# Autodesk Inventor assembly: Segway
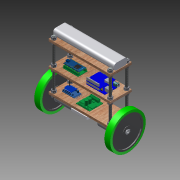
[picture p0: Inventor's stored thumbnail of the model, 180x180]
Saved by Autodesk Inventor 2012 (Build 160160000, 160)
## iProperties
Created: 2012-02-28
Part Number: Segway
Document SubType Name: Assembly
Designer: Grailas
Author: Grailas
## Documents named in this file (24)
- C:\Users\Lauszus\Documents\My Dropbox\Segway\Segway_3DModel\Segway.iam
- C:\Users\Lauszus\Documents\My Dropbox\Segway\Segway_3DModel\plate.ipt
- C:\Users\Lauszus\Documents\My Dropbox\Segway\Segway_3DModel\Screw bar.ipt
- C:\Users\Lauszus\Documents\My Dropbox\Segway\Segway_3DModel\washer.ipt
- C:\Users\Lauszus\Documents\My Dropbox\Segway\Segway_3DModel\bolt.ipt
- C:\Users\Lauszus\Documents\My Dropbox\Segway\Segway_3DModel\Imported Components\uno-assy\uno-assy.iam
- C:\Users\Lauszus\Documents\My Dropbox\Segway\Segway_3DModel\Imported Components\uno-pcb\uno-pcbEDIT.ipt
- C:\Users\Lauszus\Documents\My Dropbox\Segway\Segway_3DModel\Imported Components\C-0534237-04-3\C-0534237-04-3.ipt
- C:\Users\Lauszus\Documents\My Dropbox\Segway\Segway_3DModel\Imported Components\C-0534237-06-3\C-0534237-06-3.ipt
- C:\Users\Lauszus\Documents\My Dropbox\Segway\Segway_3DModel\usb host con.ipt
- C:\Users\Lauszus\Documents\My Dropbox\Segway\Segway_3DModel\wheel.ipt
- C:\Users\Lauszus\Documents\My Dropbox\Segway\Segway_3DModel\Hub.ipt
- C:\Users\Lauszus\Documents\My Dropbox\Segway\Segway_3DModel\bracket.ipt
- C:\Users\Lauszus\Documents\My Dropbox\Segway\Segway_3DModel\motor.ipt
- C:\Users\Lauszus\Documents\My Dropbox\Segway\Segway_3DModel\battery.ipt
- C:\Users\Lauszus\Documents\My Dropbox\Segway\Segway_3DModel\Imported Components\MBedPCB\MBedPCB.ipt
- C:\Users\Lauszus\Documents\My Dropbox\Segway\Segway_3DModel\snap ring.ipt
- C:\Users\Lauszus\Documents\My Dropbox\Segway\Segway_3DModel\Motorcontroller.ipt
- C:\Users\Lauszus\Documents\My Dropbox\Segway\Segway_3DModel\Breadboard.ipt
- C:\Users\Lauszus\Documents\My Dropbox\Segway\Segway_3DModel\Breadboard_parts.ipt
- C:\Users\Lauszus\Documents\My Dropbox\Segway\Segway_3DModel\IMU.ipt
- C:\Users\Lauszus\Documents\My Dropbox\Segway\Segway_3DModel\Adafruit xbee adapter.ipt
- C:\Users\Lauszus\Documents\My Dropbox\Segway\Segway_3DModel\mbed breakout board.ipt
- C:\Users\Lauszus\Documents\My Dropbox\Segway\Segway_3DModel\XBee_edit.ipt
## Components (81 placed, 23 different names)
1. plate:1 — Insert:1, Insert:2, Insert:4, Insert:5, Insert:6, Insert:7, Insert:8, Insert:9, Mate:5, Insert:13, Insert:15, Insert:17, Insert:19, Mate:28, Flush:11, Mate:30, Mate:31, Flush:12, Mate:36, Mate:52, Mate:65, Flush:15, Mate:67, Flush:19, Mate:70, Flush:20
2. Screw bar:1 — Insert:4, Mate:3, Mate:6
3. Screw bar:2 — Insert:5, Mate:1, Mate:8
4. Screw bar:3 — Insert:1, Mate:4, Mate:7
5. Screw bar:4 — Insert:6, Mate:2, Mate:9
6. washer:1 — Insert:2, Insert:3
7. washer:2 — Insert:7, Insert:10
8. washer:3 — Insert:8, Insert:11, Mate:52
9. washer:4 — Insert:9, Insert:12
10. bolt:1 — Insert:3
11. bolt:2 — Insert:10
12. bolt:3 — Insert:11
13. bolt:4 — Insert:12
14. washer:5 — Insert:19, Insert:20
15. washer:6 — Insert:21, Insert:23
16. washer:7 — Insert:26, Insert:28
17. washer:8 — Insert:25, Insert:27
18. bolt:5 — Insert:23
19. bolt:6 — Insert:14
20. bolt:7 — Insert:16
21. bolt:8 — Insert:18
22. bolt:9 — Insert:24
23. bolt:10 — Insert:20
24. bolt:11 — Insert:27
25. bolt:12 — Insert:28
26. washer:9 — Insert:15, Insert:16
27. washer:10 — Insert:22, Insert:24
28. washer:11 — Insert:17, Insert:18
29. washer:12 — Insert:13, Insert:14
30. plate:2 — Mate:1, Mate:2, Mate:3, Mate:4, Mate:5, Insert:21, Insert:22, Insert:25, Insert:26, Insert:29, Insert:31, Insert:33, Insert:35, Mate:10, Mate:11, Flush:1, Mate:13, Angle:2, Mate:72, Flush:23, Flush:24
31. plate:3 — Mate:6, Mate:7, Mate:8, Mate:9, Insert:37, Insert:38, Insert:41, Insert:42, Mate:10, Insert:45, Insert:46, Insert:47, Insert:48, Mate:50, Flush:13, Flush:14
32. washer:13 — Insert:33, Insert:34
33. washer:14 — Insert:31, Insert:32
34. washer:15 — Insert:29, Insert:30
35. washer:16 — Insert:35, Insert:36
36. bolt:13 — Insert:32
37. bolt:14 — Insert:36
38. bolt:15 — Insert:34
39. bolt:16 — Insert:30
40. bolt:17 — Insert:39
41. bolt:18 — Insert:40
42. bolt:19 — Insert:43
43. bolt:20 — Insert:44
44. washer:17 — Insert:37, Insert:39
45. washer:18 — Insert:38, Insert:40
46. washer:19 — Insert:41, Insert:43
47. washer:20 — Insert:42, Insert:44
48. washer:21 — Insert:47, Insert:52
49. washer:22 — Insert:48, Insert:49
50. washer:23 — Insert:46, Insert:50
51. washer:24 — Insert:45, Insert:51
52. bolt:21 — Insert:51
53. bolt:22 — Insert:52
54. bolt:23 — Insert:49
55. bolt:24 — Insert:50
56. uno-assy:1 [sub-assembly] — Mate:11, Flush:1, Mate:12, Angle:1, Mate:15, Flush:2, Flush:3, Flush:4, Flush:7
57. uno-pcbEDIT:1 — Mate:15, Flush:2, Flush:3, Mate:16, Mate:17, Mate:18, Mate:19, Mate:20, Mate:21, Mate:22, Mate:23, Mate:24, Mate:25, Mate:26
58. C-0534237-04-3:1 — Flush:5, Mate:18, Mate:19
59. C-0534237-04-3:2 — Mate:16, Mate:17, Flush:4, Flush:5
60. C-0534237-06-3:1 — Mate:20, Mate:22, Flush:6, Flush:7
61. C-0534237-06-3:2 — Mate:21, Mate:23, Flush:6
62. usb host con:1 — Mate:24, Mate:25, Mate:26
63. bracket:1 — Flush:12, Mate:36, Mate:37, Mate:38, Mate:39, Insert:57, Insert:58
64. bracket:2 — Mate:28, Flush:11, Mate:32, Mate:33, Mate:34, Insert:55, Insert:56
65. motor:1 — Insert:57, Insert:58, Insert:59
66. motor:2 — Insert:55, Insert:56, Insert:62
67. wheel:1 — Insert:60, Mate:75
68. Hub:1 — Insert:59, Insert:60, Mate:75, Insert:61
69. wheel:2 — Insert:63, Mate:76
70. Hub:2 — Insert:62, Insert:63, Mate:76, Insert:64
71. battery:1 — Mate:50, Flush:13, Flush:14
72. MBedPCB:1 — Mate:73, Flush:25, Flush:26
73. snap ring:1 — Insert:61
74. snap ring:2 — Insert:64
75. Motorcontroller:1 — Mate:65, Flush:15
76. Breadboard:1 — Mate:67, Mate:68, Flush:17, Mate:69, Flush:18, Flush:19
77. Breadboard_parts:1 — Mate:68, Flush:17
78. IMU:1 — Mate:69, Flush:18
79. Adafruit xbee adapter:1 — Mate:70, Flush:20, Mate:74, Flush:27, Flush:28
80. mbed breakout board:1 — Mate:72, Flush:23, Flush:24, Mate:73, Flush:25, Flush:26
81. XBee_edit:1 — Mate:74, Flush:27, Flush:28
## Relationships (136: Insert 62, Mate 50, Flush 22, Angle 2)
- Insert:1 (-7 mm): plate:1 ↔ Screw bar:3
- Insert:2: plate:1 ↔ washer:1
- Insert:3: washer:1 ↔ bolt:1
- Insert:4 (-7 mm): plate:1 ↔ Screw bar:1
- Insert:5 (-7 mm): plate:1 ↔ Screw bar:2
- Insert:6 (-7 mm): plate:1 ↔ Screw bar:4
- Insert:7: plate:1 ↔ washer:2
- Insert:8: plate:1 ↔ washer:3
- Insert:9: plate:1 ↔ washer:4
- Insert:10: washer:2 ↔ bolt:2
- Insert:11: washer:3 ↔ bolt:3
- Insert:12: washer:4 ↔ bolt:4
- Mate:1: Screw bar:2 ↔ plate:2
- Mate:2: Screw bar:4 ↔ plate:2
- Mate:3: Screw bar:1 ↔ plate:2
- Mate:4: Screw bar:3 ↔ plate:2
- Mate:5 (70 mm): plate:1 ↔ plate:2
- Insert:13: plate:1 ↔ washer:12
- Insert:14: bolt:6 ↔ washer:12
- Insert:15: plate:1 ↔ washer:9
- Insert:16: bolt:7 ↔ washer:9
- Insert:17: plate:1 ↔ washer:11
- Insert:18: bolt:8 ↔ washer:11
- Insert:19: plate:1 ↔ washer:5
- Insert:20: washer:5 ↔ bolt:10
- Insert:21: washer:6 ↔ plate:2
- Insert:22: washer:10 ↔ plate:2
- Insert:23: washer:6 ↔ bolt:5
- Insert:24: bolt:9 ↔ washer:10
- Insert:25: washer:8 ↔ plate:2
- Insert:26: washer:7 ↔ plate:2
- Insert:27: washer:8 ↔ bolt:11
- Insert:28: washer:7 ↔ bolt:12
- Insert:29: plate:2 ↔ washer:15
- Insert:30: washer:15 ↔ bolt:16
- Insert:31: plate:2 ↔ washer:14
- Insert:32: washer:14 ↔ bolt:13
- Insert:33: plate:2 ↔ washer:13
- Insert:34: washer:13 ↔ bolt:15
- Insert:35: plate:2 ↔ washer:16
- Insert:36: washer:16 ↔ bolt:14
- Mate:6: Screw bar:1 ↔ plate:3
- Mate:7: Screw bar:3 ↔ plate:3
- Mate:8: Screw bar:2 ↔ plate:3
- Mate:9: Screw bar:4 ↔ plate:3
- Insert:37: plate:3 ↔ washer:17
- Insert:38: plate:3 ↔ washer:18
- Insert:39: bolt:17 ↔ washer:17
- Insert:40: bolt:18 ↔ washer:18
- Insert:41: plate:3 ↔ washer:19
- Insert:42: plate:3 ↔ washer:20
- Insert:43: bolt:19 ↔ washer:19
- Insert:44: bolt:20 ↔ washer:20
- Mate:10 (75 mm): plate:2 ↔ plate:3
- Insert:45: plate:3 ↔ washer:24
- Insert:46: plate:3 ↔ washer:23
- Insert:47: plate:3 ↔ washer:21
- Insert:48: plate:3 ↔ washer:22
- Insert:49: washer:22 ↔ bolt:23
- Insert:50: washer:23 ↔ bolt:24
- Insert:51: washer:24 ↔ bolt:21
- Insert:52: washer:21 ↔ bolt:22
- Mate:11: plate:2 ↔ uno-assy:1
- Flush:1 (30 mm): plate:2 ↔ uno-assy:1
- Mate:12: uno-assy:1
- Angle:1 (0 deg): uno-assy:1
- Mate:13: plate:2
- Angle:2 (0 deg): plate:2
- Mate:14
- Mate:15: uno-assy:1 ↔ uno-pcbEDIT:1
- Flush:2: uno-assy:1 ↔ uno-pcbEDIT:1
- Flush:3: uno-assy:1 ↔ uno-pcbEDIT:1
- Mate:16: uno-pcbEDIT:1 ↔ C-0534237-04-3:2
- Mate:17: uno-pcbEDIT:1 ↔ C-0534237-04-3:2
- Flush:4: uno-assy:1 ↔ C-0534237-04-3:2
- Flush:5: C-0534237-04-3:1 ↔ C-0534237-04-3:2
- Mate:18: uno-pcbEDIT:1 ↔ C-0534237-04-3:1
- Mate:19: uno-pcbEDIT:1 ↔ C-0534237-04-3:1
- Mate:20: uno-pcbEDIT:1 ↔ C-0534237-06-3:1
- Mate:21: uno-pcbEDIT:1 ↔ C-0534237-06-3:2
- Mate:22: uno-pcbEDIT:1 ↔ C-0534237-06-3:1
- Mate:23: uno-pcbEDIT:1 ↔ C-0534237-06-3:2
- Flush:6: C-0534237-06-3:1 ↔ C-0534237-06-3:2
- Flush:7: uno-assy:1 ↔ C-0534237-06-3:1
- Mate:24: uno-pcbEDIT:1 ↔ usb host con:1
- Mate:25 (14 mm): uno-pcbEDIT:1 ↔ usb host con:1
- Mate:26 (2 mm): uno-pcbEDIT:1 ↔ usb host con:1
- Mate:28: plate:1 ↔ bracket:2
- Flush:11: plate:1 ↔ bracket:2
- Mate:30: plate:1
- Mate:31: plate:1
- Mate:32: bracket:2
- Mate:33: bracket:2
- Mate:34: bracket:2
- Mate:35
- Flush:12: plate:1 ↔ bracket:1
- Mate:36: plate:1 ↔ bracket:1
- Mate:37: bracket:1
- Mate:38: bracket:1
- Mate:39: bracket:1
- Mate:40
- Insert:55: bracket:2 ↔ motor:2
- Insert:56: bracket:2 ↔ motor:2
- Insert:57: bracket:1 ↔ motor:1
- Insert:58: bracket:1 ↔ motor:1
- Mate:50: plate:3 ↔ battery:1
- Flush:13 (1.5 mm): plate:3 ↔ battery:1
- Flush:14 (14.5 mm): plate:3 ↔ battery:1
- Mate:52: plate:1 ↔ washer:3
- Mate:65: plate:1 ↔ Motorcontroller:1
- Flush:15 (83.893 mm): plate:1 ↔ Motorcontroller:1
- Mate:67: plate:1 ↔ Breadboard:1
- Mate:68: Breadboard:1 ↔ Breadboard_parts:1
- Flush:17 (5 mm): Breadboard:1 ↔ Breadboard_parts:1
- Mate:69: Breadboard:1 ↔ IMU:1
- Flush:18 (1 mm): Breadboard:1 ↔ IMU:1
- Flush:19 (-4 mm): plate:1 ↔ Breadboard:1
- Mate:70: plate:1 ↔ Adafruit xbee adapter:1
- Flush:20 (-24.303 mm): plate:1 ↔ Adafruit xbee adapter:1
- Mate:72: plate:2 ↔ mbed breakout board:1
- Flush:23 (30 mm): plate:2 ↔ mbed breakout board:1
- Flush:24 (22.8895 mm): plate:2 ↔ mbed breakout board:1
- Mate:73 (10 mm): MBedPCB:1 ↔ mbed breakout board:1
- Flush:25 (-0.8 mm): MBedPCB:1 ↔ mbed breakout board:1
- Flush:26 (1.5 mm): MBedPCB:1 ↔ mbed breakout board:1
- Mate:74 (5 mm): Adafruit xbee adapter:1 ↔ XBee_edit:1
- Flush:27 (0.1 mm): Adafruit xbee adapter:1 ↔ XBee_edit:1
- Flush:28 (0.5 mm): Adafruit xbee adapter:1 ↔ XBee_edit:1
- Insert:59: motor:1 ↔ Hub:1
- Insert:60: wheel:1 ↔ Hub:1
- Mate:75: wheel:1 ↔ Hub:1
- Insert:61: Hub:1 ↔ snap ring:1
- Insert:62: motor:2 ↔ Hub:2
- Insert:63: wheel:2 ↔ Hub:2
- Mate:76: wheel:2 ↔ Hub:2
- Insert:64: Hub:2 ↔ snap ring:2
